# Autodesk Inventor assembly: DriveTrainSides
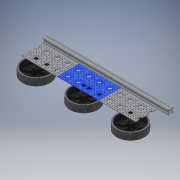
[picture p0: Inventor's stored thumbnail of the model, 180x180]
Saved by Autodesk Inventor 2018 (Build 220112000, 112)
## iProperties
Created: 2017-10-27
Part Number: DriveTrainSides
Document SubType Name: Assembly
Designer: ball
Author: ball
## Documents named in this file (5)
- C:\FTC\2017Robot\wheels.iam
- C:\FTC\Andymark\am-2648_4inWheel8mmHub.ipt
- C:\FTC\Actobotics\565 parts\565062.ipt
- C:\FTC\Actobotics\585 parts\585002_5_25x3_0.ipt
- C:\FTC\Actobotics\585 parts\585002_6_0x3_0.ipt
## Components (7 placed, 4 different names)
1. am-2648_4inWheel8mmHub:1 — Mate:3, Mate:4
2. am-2648_4inWheel8mmHub:2 — Mate:5, Mate:6
3. am-2648_4inWheel8mmHub:3 — Mate:7, Mate:8
4. 565062:1 — Mate:9, Flush:1
5. 585002_5_25x3_0:1 — Mate:1, Mate:3, Mate:4
6. 585002_5_25x3_0:2 — Mate:2, Mate:7, Mate:8, Mate:9, Flush:1
7. 585002_6_0x3_0:1 — Mate:1, Mate:2, Mate:5, Mate:6
## Relationships (10: Mate 9, Flush 1)
- Mate:1: 585002_5_25x3_0:1 ↔ 585002_6_0x3_0:1
- Mate:2: 585002_5_25x3_0:2 ↔ 585002_6_0x3_0:1
- Mate:3: am-2648_4inWheel8mmHub:1 ↔ 585002_5_25x3_0:1
- Mate:4 (25.4 mm): am-2648_4inWheel8mmHub:1 ↔ 585002_5_25x3_0:1
- Mate:5: am-2648_4inWheel8mmHub:2 ↔ 585002_6_0x3_0:1
- Mate:6 (25.4 mm): am-2648_4inWheel8mmHub:2 ↔ 585002_6_0x3_0:1
- Mate:7: am-2648_4inWheel8mmHub:3 ↔ 585002_5_25x3_0:2
- Mate:8 (25.4 mm): am-2648_4inWheel8mmHub:3 ↔ 585002_5_25x3_0:2
- Mate:9: 565062:1 ↔ 585002_5_25x3_0:2
- Flush:1 (-19.05 mm): 565062:1 ↔ 585002_5_25x3_0:2
